# Autodesk Inventor assembly: CYC_limitswitch assembly
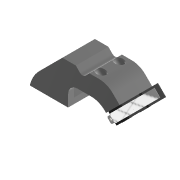
[picture p0: Inventor's stored thumbnail of the model, 180x180]
Saved by Autodesk Inventor 2020.3 (Build 243373000, 373)
## iProperties
Created: 2021-10-18
Part Number: CYC_limitswitch assembly
Document SubType Name: Assembly
Designer: justi
Author: justi
## Documents named in this file (3)
- F:\UQ Engineering\2021 ~ 5th Year\Semester 2\METR4911-THESIS\FarmBot CAD\FarmBotV1\CYC_limitswitch assembly.iam
- F:\UQ Engineering\2021 ~ 5th Year\Semester 2\METR4911-THESIS\FarmBot CAD\FarmBotV1\CYC_LimitSwitchMount.ipt
- F:\UQ Engineering\2021 ~ 5th Year\Semester 2\METR4911-THESIS\FarmBot CAD\FarmBotV1\limitswitch.ipt
## Components (2 placed, 2 different names)
1. CYC_LimitSwitchMount:1 — Mate:1, Mate:2, Mate:3, Mate:4
2. limitswitch:1 — Mate:2, Mate:3, Mate:4
## Relationships (4: Mate 4)
- Mate:1: CYC_LimitSwitchMount:1
- Mate:2: CYC_LimitSwitchMount:1 ↔ limitswitch:1
- Mate:3: CYC_LimitSwitchMount:1 ↔ limitswitch:1
- Mate:4: CYC_LimitSwitchMount:1 ↔ limitswitch:1
